# Autodesk Inventor assembly: FOR STRINGING ILLUSTRATION
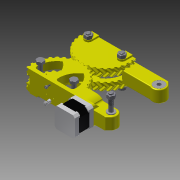
[picture p0: Inventor's stored thumbnail of the model, 180x180]
Saved by Autodesk Inventor 2013 (Build 170138000, 138)
## iProperties
Created: 2013-12-02
Part Number: FOR STRINGING ILLUSTRATION
Document SubType Name: Assembly
Designer: employee
Author: employee
## Documents named in this file (3)
- C:\Users\employee\Desktop\ConceptFORGE\ConceptFORGE\GUS Simpson\INVENTOR FILES\FOR STRINGING ILLUSTRATION.iam
- C:\Users\employee\Desktop\ConceptFORGE\ConceptFORGE\GUS Simpson\INVENTOR FILES\MOTOR ARM.iam
- C:\Users\employee\Desktop\ConceptFORGE\ConceptFORGE\GUS Simpson\INVENTOR FILES\SLAVE ARM.iam
## Components (2 placed, 2 different names)
1. MOTOR ARM:1 [sub-assembly] — Flush:1, Angle:1, Mate:1, Mate:2
2. SLAVE ARM:1 [sub-assembly] — Flush:1, Angle:1, Mate:1, Mate:2
## Relationships (4: Mate 2, Flush 1, Angle 1)
- Flush:1: MOTOR ARM:1 ↔ SLAVE ARM:1
- Angle:1 (0 deg): MOTOR ARM:1 ↔ SLAVE ARM:1
- Mate:1 (100 mm): MOTOR ARM:1 ↔ SLAVE ARM:1
- Mate:2 (75 mm): MOTOR ARM:1 ↔ SLAVE ARM:1
